# Autodesk Inventor assembly: ASY ДМФ 0100 Барабан v2.1
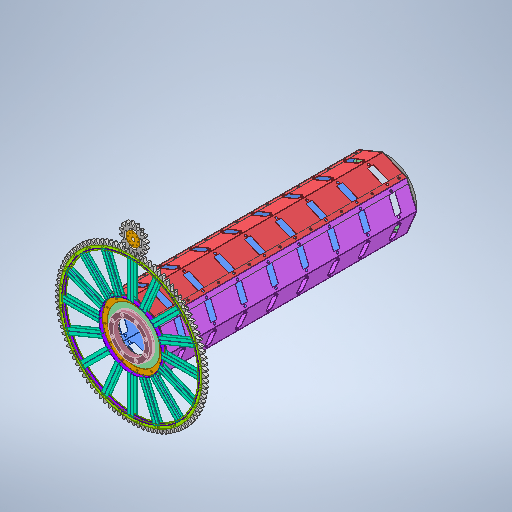
[picture p0: Inventor's stored thumbnail of the model, 512x512]
Saved by Autodesk Inventor 2025 (Build 290162010, 162A)
## iProperties
Created: 2024-04-28
Part Number: ASY ДМФ 0100 Барабан v2.1
Document SubType Name: Assembly
Designer: pokla
Author: pokla
## Documents named in this file (22)
- C:\Users\pokla\Documents\Inventor\ДФО\ДМФ\DMF-Disk-Micro-Filter\Барабан v2.1\ASY ДМФ 0100 Барабан v2.1.iam
- C:\Users\pokla\Documents\Inventor\ДФО\ДМФ\DMF-Disk-Micro-Filter\Барабан v2.1\DMF 01 21 Барабан торец НОС v2.1.ipt
- C:\Users\pokla\Documents\Inventor\ДФО\ДМФ\DMF-Disk-Micro-Filter\Барабан v2.1\DMF 01 13 Барабан Лист лев брт v2.1.ipt
- C:\Users\pokla\Documents\Inventor\ДФО\ДМФ\DMF-Disk-Micro-Filter\Барабан v2.1\DMF 01 14 Барабан Лист прав брт v2.1.ipt
- C:\Users\pokla\Documents\Inventor\ДФО\ДМФ\DMF-Disk-Micro-Filter\Барабан v2.1\DMF 01 31 Барабан Опорное кольцо НОС v2.1.ipt
- C:\Users\pokla\Documents\Inventor\ДФО\ДМФ\DMF-Disk-Micro-Filter\Барабан v2.1\DMF 01 17 опора крышки v2.1.ipt
- C:\Users\pokla\Documents\Inventor\ДФО\ДМФ\DMF-Disk-Micro-Filter\Барабан v2.1\DMF 000 размеры v2.1.ipt
- C:\Users\pokla\Documents\Inventor\ДФО\ДМФ\DMF-Disk-Micro-Filter\Барабан v2.1\DMF 01 12 Барабан усилитель v2.1.ipt
- C:\Users\pokla\Documents\Inventor\ДФО\ДМФ\DMF-Disk-Micro-Filter\Барабан v2.1\ASY DMF 010 cap v2.1.iam
- C:\Users\pokla\Documents\Inventor\ДФО\ДМФ\DMF-Disk-Micro-Filter\Барабан v2.1\DMF 01 32 Барабан Опорное кольцо КОРМА v2.1.ipt
- C:\Users\pokla\Documents\Inventor\ДФО\ДМФ\DMF-Disk-Micro-Filter\Барабан v2.1\DMF 01 22 Барабан торец КОРМА v2.1.ipt
- C:\Users\pokla\Documents\Inventor\ДФО\ДМФ\DMF-Disk-Micro-Filter\Барабан v2.1\ASY DMF filter package v2.1.iam
- C:\Users\pokla\Documents\Inventor\ДФО\ДМФ\DMF-Disk-Micro-Filter\Барабан v2.1\DMF 01 21 cylinder butt end nose.ipt
- C:\Users\pokla\Documents\Inventor\ДФО\ДМФ\DMF-Disk-Micro-Filter\Барабан v2.1\DMF 2.1 01 42 Gear way 2.ipt
- C:\Users\pokla\Documents\Inventor\ДФО\ДМФ\DMF-Disk-Micro-Filter\Барабан v2.1\DMF 2.1 01 43 Gear rim 3.ipt
- C:\Users\pokla\Documents\Inventor\ДФО\ДМФ\DMF-Disk-Micro-Filter\Барабан v2.1\DMF 2.1 01 44 Gear rim 4.ipt
- C:\Users\pokla\Documents\Inventor\ДФО\ДМФ\DMF-Disk-Micro-Filter\Барабан v2.1\DMF 2.1 01 45 Gear ring 5.ipt
- C:\Users\pokla\Documents\Inventor\ДФО\ДМФ\DMF-Disk-Micro-Filter\Барабан v2.1\DMF 2.1 01 46 Gear axis wheel 6.ipt
- C:\Users\pokla\Documents\Inventor\ДФО\ДМФ\DMF-Disk-Micro-Filter\Барабан v2.1\DMF 01 13 Барабан усилитель v2.1.ipt
- C:\Users\pokla\Documents\Inventor\ДФО\ДМФ\DMF-Disk-Micro-Filter\Барабан v2.1\DMF small gear.ipt
- C:\Users\pokla\Documents\Inventor\ДФО\ДМФ\DMF-Disk-Micro-Filter\Барабан v2.1\DMF flange small gear.ipt
- C:\Users\pokla\Documents\Inventor\ДФО\ДМФ\DMF-Disk-Micro-Filter\шестерни 06.09.2025\DMF sector big gear 2.1.ipt
## Components (106 placed, 21 different names)
1. DMF 000 размеры v2.1.ipt:1 — Rigid:30
2. DMF 01 21 Барабан торец НОС v2.1.ipt:1 — Mate:15, Flush:8, Flush:9, Flush:10, Flush:11, Mate:16, Mate:17, Mate:19, Mate:21, Flush:15, Flush:16, Flush:17, Mate:23, Rigid:27, Rigid:29, Rigid:30, Rigid:34
3. DMF 01 31 Барабан Опорное кольцо НОС v2.1.ipt:1 — Rigid:29
4. DMF 01 32 Барабан Опорное кольцо КОРМА v2.1.ipt:1 — Rigid:20
5. DMF 01 22 Барабан торец КОРМА v2.1.ipt:1 — Flush:12, Flush:13, Mate:18, Rigid:20
6. DMF 01 13 Барабан Лист лев брт v2.1.ipt:1 — Flush:10, Flush:11, Mate:16, Flush:13, Mate:18, Mate:20, Mate:29
7. DMF 01 14 Барабан Лист прав брт v2.1.ipt:1 — Flush:8, Flush:9, Mate:17, Flush:12, Mate:22, Mate:28
8. DMF 01 17 опора крышки v2.1.ipt:1 — Mate:21, Flush:15, Mate:22
9. DMF 01 17 опора крышки v2.1.ipt:2 — Mate:19, Mate:20, Mate:27
10. ASY DMF 010 cap v2.1.iam:1 [sub-assembly] — Flush:16, Flush:17, Mate:23, Mate:27
11. DMF 01 21 cylinder butt end nose.ipt:1 — Mate:28, Mate:29
12. DMF 2.1 01 45 Gear ring 5.ipt:1 — Rigid:21, Rigid:22, Rigid:23, Rigid:27, Rigid:31
13. DMF 2.1 01 46 Gear axis wheel 6.ipt:1 — Rigid:31
14. DMF small gear.ipt:1 — Rigid:33
15. DMF flange small gear.ipt:1 — Rigid:33
16. ASY DMF filter package v2.1.iam:1 [sub-assembly] — Mate:24, Mate:25
17. ASY DMF filter package v2.1.iam:2 [sub-assembly]
18. ASY DMF filter package v2.1.iam:3 [sub-assembly]
19. ASY DMF filter package v2.1.iam:4 [sub-assembly]
20. ASY DMF filter package v2.1.iam:5 [sub-assembly]
21. ASY DMF filter package v2.1.iam:6 [sub-assembly]
22. ASY DMF filter package v2.1.iam:7 [sub-assembly]
23. ASY DMF filter package v2.1.iam:8 [sub-assembly]
24. DMF 2.1 01 43 Gear rim 3.ipt:1 — Rigid:24
25. DMF 2.1 01 43 Gear rim 3.ipt:2 — Rigid:23, Rigid:24
26. DMF 2.1 01 43 Gear rim 3.ipt:3
27. DMF 2.1 01 43 Gear rim 3.ipt:4
28. DMF 2.1 01 43 Gear rim 3.ipt:5
29. DMF 2.1 01 43 Gear rim 3.ipt:6
30. DMF 2.1 01 43 Gear rim 3.ipt:7
31. DMF 2.1 01 43 Gear rim 3.ipt:8
32. DMF 2.1 01 44 Gear rim 4.ipt:1 — Rigid:22
33. DMF 2.1 01 44 Gear rim 4.ipt:2
34. DMF 2.1 01 44 Gear rim 4.ipt:3
35. DMF 01 12 Барабан усилитель v2.1.ipt:1 — Mate:30, Tangent:1, Mate:31, Rigid:21, Flush:18, Mate:32, Mate:33
36. DMF 2.1 01 42 Gear way 2.ipt:1 — Mate:30, Tangent:1, Mate:31
37. DMF 01 13 Барабан усилитель v2.1.ipt:1 — Flush:18, Mate:32, Mate:33
38. DMF 01 12 Барабан усилитель v2.1.ipt:2
39. DMF 2.1 01 42 Gear way 2.ipt:2
40. DMF 01 13 Барабан усилитель v2.1.ipt:2
41. DMF 01 12 Барабан усилитель v2.1.ipt:3
42. DMF 2.1 01 42 Gear way 2.ipt:3
43. DMF 01 13 Барабан усилитель v2.1.ipt:3
44. DMF 01 12 Барабан усилитель v2.1.ipt:4
45. DMF 2.1 01 42 Gear way 2.ipt:4
46. DMF 01 13 Барабан усилитель v2.1.ipt:4
47. DMF 01 12 Барабан усилитель v2.1.ipt:5
48. DMF 2.1 01 42 Gear way 2.ipt:5
49. DMF 01 13 Барабан усилитель v2.1.ipt:5
50. DMF 01 12 Барабан усилитель v2.1.ipt:6
51. DMF 2.1 01 42 Gear way 2.ipt:6
52. DMF 01 13 Барабан усилитель v2.1.ipt:6
53. DMF 01 12 Барабан усилитель v2.1.ipt:7
54. DMF 2.1 01 42 Gear way 2.ipt:7
55. DMF 01 13 Барабан усилитель v2.1.ipt:7
56. DMF 01 12 Барабан усилитель v2.1.ipt:8
57. DMF 2.1 01 42 Gear way 2.ipt:8
58. DMF 01 13 Барабан усилитель v2.1.ipt:8
59. DMF 01 12 Барабан усилитель v2.1.ipt:9
60. DMF 2.1 01 42 Gear way 2.ipt:9
61. DMF 01 13 Барабан усилитель v2.1.ipt:9
62. DMF 01 12 Барабан усилитель v2.1.ipt:10
63. DMF 2.1 01 42 Gear way 2.ipt:10
64. DMF 01 13 Барабан усилитель v2.1.ipt:10
65. DMF 01 12 Барабан усилитель v2.1.ipt:11
66. DMF 2.1 01 42 Gear way 2.ipt:11
67. DMF 01 13 Барабан усилитель v2.1.ipt:11
68. DMF 01 12 Барабан усилитель v2.1.ipt:12
69. DMF 2.1 01 42 Gear way 2.ipt:12
70. DMF 01 13 Барабан усилитель v2.1.ipt:12
71. DMF 01 12 Барабан усилитель v2.1.ipt:13
72. DMF 2.1 01 42 Gear way 2.ipt:13
73. DMF 01 13 Барабан усилитель v2.1.ipt:13
74. DMF 01 12 Барабан усилитель v2.1.ipt:14
75. DMF 2.1 01 42 Gear way 2.ipt:14
76. DMF 01 13 Барабан усилитель v2.1.ipt:14
77. DMF 01 12 Барабан усилитель v2.1.ipt:15
78. DMF 2.1 01 42 Gear way 2.ipt:15
79. DMF 01 13 Барабан усилитель v2.1.ipt:15
80. DMF 01 12 Барабан усилитель v2.1.ipt:16
81. DMF 2.1 01 42 Gear way 2.ipt:16
82. DMF 01 13 Барабан усилитель v2.1.ipt:16
83. DMF sector big gear 2.1.ipt:1 — Rigid:34
84. DMF sector big gear 2.1.ipt:2
85. DMF sector big gear 2.1.ipt:3
86. DMF sector big gear 2.1.ipt:4
87. DMF sector big gear 2.1.ipt:5
88. DMF sector big gear 2.1.ipt:6
89. DMF sector big gear 2.1.ipt:7
90. DMF sector big gear 2.1.ipt:8
91. DMF sector big gear 2.1.ipt:9
92. DMF sector big gear 2.1.ipt:10
93. DMF sector big gear 2.1.ipt:11
94. DMF sector big gear 2.1.ipt:12
95. DMF sector big gear 2.1.ipt:13
96. DMF sector big gear 2.1.ipt:14
97. DMF sector big gear 2.1.ipt:15
98. DMF sector big gear 2.1.ipt:16
99. DMF sector big gear 2.1.ipt:17
100. DMF sector big gear 2.1.ipt:18
101. DMF sector big gear 2.1.ipt:19
102. DMF sector big gear 2.1.ipt:20
103. DMF sector big gear 2.1.ipt:21
104. DMF sector big gear 2.1.ipt:22
105. DMF sector big gear 2.1.ipt:23
106. DMF sector big gear 2.1.ipt:24
## Component patterns: (8 elements, first: ASY DMF filter package v2.1.iam:1), (4 elements, first: DMF 2.1 01 43 Gear rim 3.ipt:1 + DMF 2.1 01 43 Gear rim 3.ipt:2), (3 elements, first: DMF 2.1 01 44 Gear rim 4.ipt:1), (16 elements, first: DMF 01 12 Барабан усилитель v2.1.ipt:1 + DMF 2.1 01 42 Gear way 2.ipt:1 + DMF 01 13 Барабан усилитель v2.1.ipt:1), (24 elements, first: DMF sector big gear 2.1.ipt:1)
## Relationships (40: Mate 18, WeldJoint 11, Flush 10, Tangent 1)
- Mate:15: DMF 01 21 Барабан торец НОС v2.1.ipt:1
- Flush:8: DMF 01 21 Барабан торец НОС v2.1.ipt:1 ↔ DMF 01 14 Барабан Лист прав брт v2.1.ipt:1
- Flush:9: DMF 01 21 Барабан торец НОС v2.1.ipt:1 ↔ DMF 01 14 Барабан Лист прав брт v2.1.ipt:1
- Flush:10: DMF 01 21 Барабан торец НОС v2.1.ipt:1 ↔ DMF 01 13 Барабан Лист лев брт v2.1.ipt:1
- Flush:11: DMF 01 21 Барабан торец НОС v2.1.ipt:1 ↔ DMF 01 13 Барабан Лист лев брт v2.1.ipt:1
- Mate:16: DMF 01 21 Барабан торец НОС v2.1.ipt:1 ↔ DMF 01 13 Барабан Лист лев брт v2.1.ipt:1
- Mate:17: DMF 01 21 Барабан торец НОС v2.1.ipt:1 ↔ DMF 01 14 Барабан Лист прав брт v2.1.ipt:1
- Flush:12: DMF 01 22 Барабан торец КОРМА v2.1.ipt:1 ↔ DMF 01 14 Барабан Лист прав брт v2.1.ipt:1
- Flush:13: DMF 01 22 Барабан торец КОРМА v2.1.ipt:1 ↔ DMF 01 13 Барабан Лист лев брт v2.1.ipt:1
- Mate:18: DMF 01 22 Барабан торец КОРМА v2.1.ipt:1 ↔ DMF 01 13 Барабан Лист лев брт v2.1.ipt:1
- Mate:19: DMF 01 21 Барабан торец НОС v2.1.ipt:1 ↔ DMF 01 17 опора крышки v2.1.ipt:2
- Mate:20: DMF 01 13 Барабан Лист лев брт v2.1.ipt:1 ↔ DMF 01 17 опора крышки v2.1.ipt:2
- Mate:21: DMF 01 21 Барабан торец НОС v2.1.ipt:1 ↔ DMF 01 17 опора крышки v2.1.ipt:1
- Flush:15 (-2 mm): DMF 01 21 Барабан торец НОС v2.1.ipt:1 ↔ DMF 01 17 опора крышки v2.1.ipt:1
- Mate:22: DMF 01 14 Барабан Лист прав брт v2.1.ipt:1 ↔ DMF 01 17 опора крышки v2.1.ipt:1
- Flush:16: DMF 01 21 Барабан торец НОС v2.1.ipt:1 ↔ ASY DMF 010 cap v2.1.iam:1
- Flush:17: DMF 01 21 Барабан торец НОС v2.1.ipt:1 ↔ ASY DMF 010 cap v2.1.iam:1
- Mate:23: DMF 01 21 Барабан торец НОС v2.1.ipt:1 ↔ ASY DMF 010 cap v2.1.iam:1
- Mate:24: ASY DMF filter package v2.1.iam:1
- Mate:25: ASY DMF filter package v2.1.iam:1
- Mate:27: DMF 01 17 опора крышки v2.1.ipt:2 ↔ ASY DMF 010 cap v2.1.iam:1
- Mate:28: DMF 01 14 Барабан Лист прав брт v2.1.ipt:1 ↔ DMF 01 21 cylinder butt end nose.ipt:1
- Mate:29: DMF 01 13 Барабан Лист лев брт v2.1.ipt:1 ↔ DMF 01 21 cylinder butt end nose.ipt:1
- Rigid:20 [WeldJoint]: DMF 01 32 Барабан Опорное кольцо КОРМА v2.1.ipt:1 ↔ DMF 01 22 Барабан торец КОРМА v2.1.ipt:1
- Mate:30: DMF 01 12 Барабан усилитель v2.1.ipt:1 ↔ DMF 2.1 01 42 Gear way 2.ipt:1
- Tangent:1: DMF 01 12 Барабан усилитель v2.1.ipt:1 ↔ DMF 2.1 01 42 Gear way 2.ipt:1
- Mate:31: DMF 01 12 Барабан усилитель v2.1.ipt:1 ↔ DMF 2.1 01 42 Gear way 2.ipt:1
- Rigid:21 [WeldJoint]: DMF 2.1 01 45 Gear ring 5.ipt:1 ↔ DMF 01 12 Барабан усилитель v2.1.ipt:1
- Rigid:22 [WeldJoint]: DMF 2.1 01 45 Gear ring 5.ipt:1 ↔ DMF 2.1 01 44 Gear rim 4.ipt:1
- Rigid:23 [WeldJoint]: DMF 2.1 01 45 Gear ring 5.ipt:1 ↔ DMF 2.1 01 43 Gear rim 3.ipt:2
- Rigid:24 [WeldJoint] (25 mm): DMF 2.1 01 43 Gear rim 3.ipt:1 ↔ DMF 2.1 01 43 Gear rim 3.ipt:2
- Rigid:27 [WeldJoint]: DMF 01 21 Барабан торец НОС v2.1.ipt:1 ↔ DMF 2.1 01 45 Gear ring 5.ipt:1
- Rigid:29 [WeldJoint]: DMF 01 21 Барабан торец НОС v2.1.ipt:1 ↔ DMF 01 31 Барабан Опорное кольцо НОС v2.1.ipt:1
- Rigid:30 [WeldJoint]: DMF 000 размеры v2.1.ipt:1 ↔ DMF 01 21 Барабан торец НОС v2.1.ipt:1
- Rigid:31 [WeldJoint]: DMF 2.1 01 45 Gear ring 5.ipt:1 ↔ DMF 2.1 01 46 Gear axis wheel 6.ipt:1
- Flush:18: DMF 01 12 Барабан усилитель v2.1.ipt:1 ↔ DMF 01 13 Барабан усилитель v2.1.ipt:1
- Mate:32 (2 mm): DMF 01 12 Барабан усилитель v2.1.ipt:1 ↔ DMF 01 13 Барабан усилитель v2.1.ipt:1
- Mate:33 (27 mm): DMF 01 12 Барабан усилитель v2.1.ipt:1 ↔ DMF 01 13 Барабан усилитель v2.1.ipt:1
- Rigid:33 [WeldJoint]: DMF small gear.ipt:1 ↔ DMF flange small gear.ipt:1
- Rigid:34 [WeldJoint] (2.5 mm): DMF 01 21 Барабан торец НОС v2.1.ipt:1 ↔ DMF sector big gear 2.1.ipt:1
